# Autodesk Inventor assembly: Toggle Clamp (GH-36204-M)
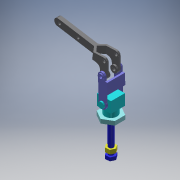
[picture p0: Inventor's stored thumbnail of the model, 180x180]
Saved by Autodesk Inventor 2019 (Build 230136000, 136)
## iProperties
Created: 2013-08-12
Part Number: Toggle Clamp (GH-36204-M)
Document SubType Name: Assembly
Designer: maste
Sending System: SolidWorks 2013
Last Author: i5-2320
Last Saved: 2015-10-23
Cfg4Qty: Default
UNIT_OF_MEASURE: - none -
code: 1 Dim myAsy As AssemblyDoc Dim myCmps Dim Cfg As String Dim CmpDoc As ModelDoc2 Dim i As Long Dim j As Long Dim cCnt As Long Dim NoUp As Long Dim myCmp As Component2 Dim tCmp As Component2 dim tm as double tm = timer Set myAsy = Assembly If Assembly.ConfigurationManager.ActiveConfiguration.Name <> Assembly.CustomInfo2("", "Cfg4Qty") Then  Assembly.Extension.ShowSmartMessage "Qtys not updated due to config", 1000, True, True  Exit Sub End If NoUp = 0 myCmps = myAsy.GetComponents(False) For i = 0 To UBound(myCmps)  Set myCmp = myCmps(i)  If (myCmp.GetSuppression = 3) Or (myCmp.Get
code2: Suppression = 2) Then   cCnt = 0   Set CmpDoc = myCmp.GetModelDoc   Cfg = myCmp.ReferencedConfiguration   For j = 0 To UBound(myCmps)    Set tCmp = myCmps(j)    If tCmp.GetSuppression <> 0 Then     If tCmp.GetModelDoc2 Is CmpDoc Then      If tCmp.ReferencedConfiguration = Cfg Then       cCnt = cCnt + 1      End If     End If    End If   Next j   CmpDoc.AddCustomInfo3 Cfg, "AutoQty", 30, ""   CmpDoc.AddCustomInfo3 Cfg, "QtyIn", 30, ""   CmpDoc.CustomInfo2(Cfg, "AutoQty") = cCnt   CmpDoc.CustomInfo2(Cfg, "QtyIn") = Assembly.GetTitle & " Cfg " & Assembly.ConfigurationManager.ActiveConfiguration.Name  Else   NoUp = NoUp + 1  End If Next i Assembly.Extension.ShowSmartMessage NoUp & " Parts not updated due to lightweight (" & timer - tm & "s)", 10000, True, True
Author: maste
## Documents named in this file (7)
- D:\Summer Drive Base V1\Summer Drivebase\GH-36204-M (PLY 38MM)\Toggle Clamp (GH-36204-M).iam
- D:\Summer Drive Base V1\Summer Drivebase\GH-36204-M (PLY 38MM)\GH-36204-M PART 1.ipt
- D:\Summer Drive Base V1\Summer Drivebase\GH-36204-M (PLY 38MM)\GH-36204-M PART 5.ipt
- D:\Summer Drive Base V1\Summer Drivebase\GH-36204-M (PLY 38MM)\GH-36204-M PART 2.ipt
- D:\Summer Drive Base V1\Summer Drivebase\GH-36204-M (PLY 38MM)\GH-36204-M PART 4.ipt
- D:\Summer Drive Base V1\Summer Drivebase\GH-36204-M (PLY 38MM)\GH-36204-M PART 6.ipt
- D:\Summer Drive Base V1\Summer Drivebase\GH-36204-M (PLY 38MM)\GH-36204-M PART 7.ipt
## Components (6 placed, 6 different names)
1. GH-36204-M PART 1:1 — Mate:3, Mate:4, Rotation:1, Mate:5, Flush:1, Rotation:2, Mate:7, Mate:8, Mate:9, Mate:10
2. GH-36204-M PART 5:1 — Mate:1, Mate:2, Mate:9, Mate:10
3. GH-36204-M PART 2:1 — Mate:1, Mate:2
4. GH-36204-M PART 4:1 — Mate:5, Flush:1, Rotation:2
5. GH-36204-M PART 6:1 — Mate:3, Mate:4, Rotation:1, Flush:2, Mate:6, Mate:7, Mate:8
6. GH-36204-M PART 7:1 — Flush:2, Mate:6
## Relationships (14: Mate 10, RelateRotation 2, Flush 2)
- Mate:1: GH-36204-M PART 5:1 ↔ GH-36204-M PART 2:1
- Mate:2: GH-36204-M PART 5:1 ↔ GH-36204-M PART 2:1
- Mate:3: GH-36204-M PART 1:1 ↔ GH-36204-M PART 6:1
- Mate:4: GH-36204-M PART 1:1 ↔ GH-36204-M PART 6:1
- Rotation:1 [RelateRotation] (1 ul): GH-36204-M PART 1:1 ↔ GH-36204-M PART 6:1
- Mate:5: GH-36204-M PART 1:1 ↔ GH-36204-M PART 4:1
- Flush:1: GH-36204-M PART 1:1 ↔ GH-36204-M PART 4:1
- Rotation:2 [RelateRotation] (1 ul): GH-36204-M PART 1:1 ↔ GH-36204-M PART 4:1
- Flush:2: GH-36204-M PART 6:1 ↔ GH-36204-M PART 7:1
- Mate:6: GH-36204-M PART 6:1 ↔ GH-36204-M PART 7:1
- Mate:7: GH-36204-M PART 1:1 ↔ GH-36204-M PART 6:1
- Mate:8: GH-36204-M PART 1:1 ↔ GH-36204-M PART 6:1
- Mate:9: GH-36204-M PART 1:1 ↔ GH-36204-M PART 5:1
- Mate:10: GH-36204-M PART 1:1 ↔ GH-36204-M PART 5:1
